# Autodesk Inventor assembly: Drive_Shaft_Assembly
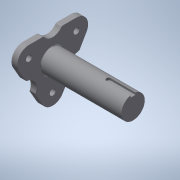
[picture p0: Inventor's stored thumbnail of the model, 180x180]
Saved by Autodesk Inventor 2021 (Build 250183000, 183)
## iProperties
Created: 2020-11-11
Part Number: Drive_Shaft_Assembly
Document SubType Name: Assembly
Designer: PhotonUser
Quantity: 1
Author: PhotonUser
## Documents named in this file (3)
- D:\PhotonUser\Downloads\Assembly Files-20201111T001656Z-001\Assembly Files\Drive_Shaft_Assembly.iam
- D:\PhotonUser\Downloads\Assembly Files-20201111T001656Z-001\Assembly Files\MotorShaft.ipt
- D:\PhotonUser\Downloads\Assembly Files-20201111T001656Z-001\Assembly Files\Torque_Triangle.ipt
## Components (2 placed, 2 different names)
1. MotorShaft:1 — Insert:1
2. Torque_Triangle:1 — Insert:1
## Relationships (1: Insert 1)
- Insert:1: MotorShaft:1 ↔ Torque_Triangle:1
